# Autodesk Inventor assembly: FE-00040-04_ASM_13_ASM
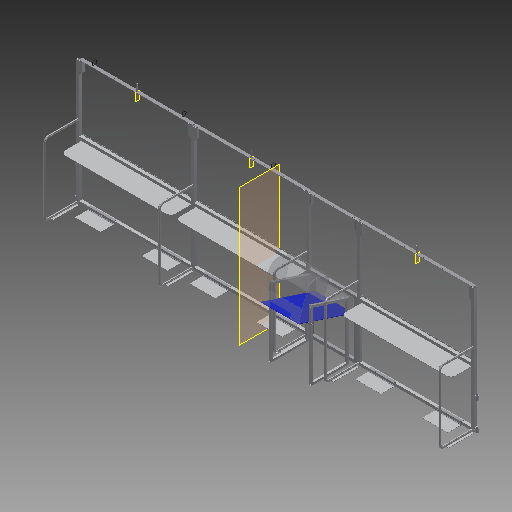
[picture p0: Inventor's stored thumbnail of the model, 512x512]
Saved by Autodesk Inventor 2017 (Build 210142000, 142)
## iProperties
Created: 2016-12-16
Part Number: FE-00040-04_ASM_13_ASM
Document SubType Name: Assembly
Designer: PhillipD
Author: PhillipD
Revision Number: 1LAST_VERSION
## Documents named in this file (10)
- C:\Users\jeff1\OneDrive\Documents\1504\217-2000-STEP\Parts\FE-00040-04_ASM_13_ASM.iam
- C:\Users\jeff1\OneDrive\Documents\1504\217-2000-STEP\Parts\FE-00002-L_ASM_2_ASM.iam
- C:\Users\jeff1\OneDrive\Documents\1504\217-2000-STEP\Parts\FE-00004_ASM_2_ASM.iam
- C:\Users\jeff1\OneDrive\Documents\1504\217-2000-STEP\Parts\FE-00001_ASM_3_ASM.iam
- C:\Users\jeff1\OneDrive\Documents\1504\217-2000-STEP\Parts\FE-00002-R_ASM_3_ASM.iam
- C:\Users\jeff1\OneDrive\Documents\1504\217-2000-STEP\Parts\FE-00007_ASM_2_ASM.iam
- C:\Users\jeff1\OneDrive\Documents\1504\217-2000-STEP\Parts\FE-00012_2.ipt
- C:\Users\jeff1\OneDrive\Documents\1504\217-2000-STEP\Parts\GE-17270_ASM_1_ASM.iam
- C:\Users\jeff1\OneDrive\Documents\1504\217-2000-STEP\Parts\PIPESTRAP_1.ipt
- C:\Users\jeff1\OneDrive\Documents\1504\217-2000-STEP\Parts\GE-17307_ASM_36_ASM_BLUE.iam
## Components (21 placed, 21 different names)
1. FE-00002-L_ASM_2_ASM_1047 [sub-assembly] — Symmetry:1
2. FE-00004_ASM_2_ASM_1048 [sub-assembly]
3. FE-00001_ASM_3_ASM_1049 [sub-assembly]
4. FE-00004_ASM_2_ASM_1050 [sub-assembly]
5. FE-00001_ASM_3_ASM_1051 [sub-assembly]
6. GE-17307_ASM_36_ASM_1052 [sub-assembly]
7. FE-00001_ASM_3_ASM_1053 [sub-assembly]
8. FE-00004_ASM_2_ASM_1054 [sub-assembly]
9. FE-00002-R_ASM_3_ASM_1055 [sub-assembly] — Symmetry:1
10. FE-00007_ASM_2_ASM_1056 [sub-assembly]
11. FE-00007_ASM_2_ASM_1057 [sub-assembly]
12. FE-00007_ASM_2_ASM_1058 [sub-assembly]
13. FE-00012_2_1059
14. FE-00012_2_1060
15. FE-00012_2_1061
16. GE-17270_ASM_1_ASM_1064 [sub-assembly]
17. GE-17270_ASM_1_ASM_1065 [sub-assembly]
18. GE-17270_ASM_1_ASM_1066 [sub-assembly]
19. PIPESTRAP_1_1067
20. PIPESTRAP_1_1068
21. PIPESTRAP_1_1069
## Relationships (1: Symmetry 1)
- Symmetry:1: FE-00002-L_ASM_2_ASM_1047 ↔ FE-00002-R_ASM_3_ASM_1055
